# Autodesk Inventor assembly: EFOI-10
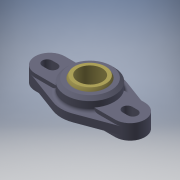
[picture p0: Inventor's stored thumbnail of the model, 180x180]
Saved by Autodesk Inventor 2017.1 (Build 211199000, 199)
## iProperties
Category: Igus Bag
Company: Autodesk, Inc.
Created: 2016-12-24
Part Number: EFOI-10
Document SubType Name: Assembly
Project: FIRST
Catalog Web Link: http://www.igus.com/wpck/5378/igubal_Flanschlager_EFOI?CL=US-en
Description: Flanged spherical bearing
Vendor: igus
Title: Flanged Spherical Bearing
Author: Autodesk, Inc.
Keywords: Gray Tote
## Documents named in this file (3)
- D:\FIRST\FIRST KOP 2017\FIRST 2017 Gray Tote\EFOI-10R.iam
- D:\FIRST\FIRST KOP 2017\FIRST 2017 Gray Tote\Parts\EFOI-10_Housing.ipt
- D:\FIRST\FIRST KOP 2017\FIRST 2017 Gray Tote\Parts\EFOI-10_Spherical Bearing.ipt
## Components (2 placed, 2 different names)
1. EFOI-10_Housing:1 — Mate:1
2. EFOI-10_Spherical Bearing:1 — Mate:1
## Relationships (1: Mate 1)
- Mate:1: EFOI-10_Housing:1 ↔ EFOI-10_Spherical Bearing:1
